# Autodesk Inventor assembly: leg_2
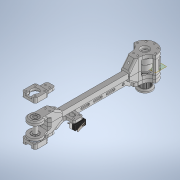
[picture p0: Inventor's stored thumbnail of the model, 180x180]
Saved by Autodesk Inventor 2020 (Build 240168000, 168)
## iProperties
Created: 2019-05-03
Part Number: leg_2
Document SubType Name: Assembly
Designer: psrob
Author: psrob
## Documents named in this file (14)
- E:\projects-2\project dog gen2\hardware\leg_bone_2.iam
- E:\projects-2\project dog gen2\hardware\bone_upper_1.ipt
- E:\projects-2\project dog gen2\hardware\bone_upper_2.ipt
- E:\projects-2\project dog gen2\hardware\bone_upper_3.ipt
- E:\projects-2\project dog gen2\hardware\bone_upper_4.ipt
- E:\projects-2\project dog gen2\hardware\bearing_4_9_4.ipt
- E:\projects-2\project dog gen2\hardware\pin_2_20.ipt
- E:\projects-2\project dog gen2\hardware\bone_upper_wheel_1.ipt
- E:\projects-2\project dog gen2\hardware\2GT_wheel.ipt
- E:\projects-2\project dog gen2\hardware\carbon_fiber_70.ipt
- E:\projects-2\project dog gen2\hardware\leg_switch_holder_1.ipt
- E:\projects-2\project dog gen2\hardware\ultra-subminiature-basic-switch-d2f-1.snapshot.2\D2F-01L.ipt
- E:\projects-2\project dog gen2\hardware\encoder_holder_down.ipt
- E:\projects-2\project dog gen2\hardware\encoder_holder_down_MIR.ipt
## Components (15 placed, 13 different names)
1. bone_upper_1:1 — Insert:1, Insert:2, Insert:8, Mate:4, Mate:5
2. bone_upper_1:2 — Insert:1, Insert:2, Insert:7, Mate:6, Insert:14, Angle:1
3. bone_upper_2:1 — Insert:3, Insert:4, Insert:6, Insert:10, Insert:11, Mate:1, Mate:3, Insert:13
4. bone_upper_3:1 — Insert:3, Insert:4, Flush:2, Insert:5, Insert:12, Mate:2
5. bone_upper_4:1 — Flush:2, Insert:5, Insert:6
6. bearing_4_9_4:1 — Insert:7, Insert:9, Insert:17
7. bearing_4_9_4:2 — Insert:8
8. pin_2_20:1 — Insert:9
9. bone_upper_wheel_1:1 — Insert:10, Insert:11
10. 2GT_wheel:1 — Insert:12
11. carbon_fiber_70:1 — Mate:1, Mate:2, Mate:3, Mate:4, Mate:5, Mate:6, Flush:3
12. leg_switch_holder_1:1 — Flush:3, Insert:13, Insert:14, Insert:15, Insert:16
13. D2F-01L:1 — Insert:15, Insert:16
14. encoder_holder_down:1 — Insert:17, Angle:1
15. encoder_holder_down_MIR:1
## Relationships (26: Insert 17, Mate 6, Flush 2, Angle 1)
- Insert:1: bone_upper_1:1 ↔ bone_upper_1:2
- Insert:2: bone_upper_1:1 ↔ bone_upper_1:2
- Insert:3: bone_upper_2:1 ↔ bone_upper_3:1
- Insert:4: bone_upper_2:1 ↔ bone_upper_3:1
- Flush:2: bone_upper_3:1 ↔ bone_upper_4:1
- Insert:5: bone_upper_3:1 ↔ bone_upper_4:1
- Insert:6: bone_upper_2:1 ↔ bone_upper_4:1
- Insert:7: bone_upper_1:2 ↔ bearing_4_9_4:1
- Insert:8: bone_upper_1:1 ↔ bearing_4_9_4:2
- Insert:9 (0.5 mm): bearing_4_9_4:1 ↔ pin_2_20:1
- Insert:10: bone_upper_2:1 ↔ bone_upper_wheel_1:1
- Insert:11: bone_upper_2:1 ↔ bone_upper_wheel_1:1
- Insert:12 (0.3 mm): bone_upper_3:1 ↔ 2GT_wheel:1
- Mate:1: bone_upper_2:1 ↔ carbon_fiber_70:1
- Mate:2: bone_upper_3:1 ↔ carbon_fiber_70:1
- Mate:3: bone_upper_2:1 ↔ carbon_fiber_70:1
- Mate:4: bone_upper_1:1 ↔ carbon_fiber_70:1
- Mate:5: bone_upper_1:1 ↔ carbon_fiber_70:1
- Mate:6: bone_upper_1:2 ↔ carbon_fiber_70:1
- Flush:3: carbon_fiber_70:1 ↔ leg_switch_holder_1:1
- Insert:13: bone_upper_2:1 ↔ leg_switch_holder_1:1
- Insert:14: bone_upper_1:2 ↔ leg_switch_holder_1:1
- Insert:15: leg_switch_holder_1:1 ↔ D2F-01L:1
- Insert:16: leg_switch_holder_1:1 ↔ D2F-01L:1
- Insert:17: bearing_4_9_4:1 ↔ encoder_holder_down:1
- Angle:1 (0 deg): bone_upper_1:2 ↔ encoder_holder_down:1
